# Autodesk Inventor assembly: 240710_case
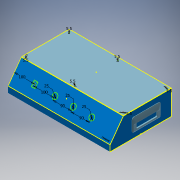
[picture p0: Inventor's stored thumbnail of the model, 180x180]
Saved by Autodesk Inventor 2016 (Build 200138000, 138)
## iProperties
Created: 2024-07-10
Part Number: 240710_case
Material: 일반
Document SubType Name: Assembly
Designer: pc
Author: pc
## Documents named in this file (5)
- D:\CAD_HCH\240710\240710_case.iam
- D:\CAD_HCH\240710\240710_part2.ipt
- D:\CAD_HCH\240710\240710_part3.ipt
- C:\Users\pc\Documents\Inventor\Content Center Files\R2016\ko-KR\ANSI B18.2.3.2M(1)\ANSI B18.2.3.2M - M5x0.8 x 8(2)8.ipt
- D:\CAD_HCH\240711\DR_A-MP200\DR_A-MP200.ipt
## Components (10 placed, 4 different names)
1. 240710_part2:1 — 메이트:1, 플러쉬:1, 플러쉬:2, 메이트:2, 메이트:3
2. 240710_part3:1 — 메이트:1, 플러쉬:1, 플러쉬:2, 삽입:1, 삽입:2, 삽입:3, 삽입:4, 삽입:5, 삽입:6
3. 6각 나사 - 미터 (1) M5x0.8 x 8:1 — 삽입:1
4. 6각 나사 - 미터 (1) M5x0.8 x 8:2 — 삽입:2
5. DR_A-MP200:1 — 메이트:2
6. DR_A-MP200:2 — 메이트:3
7. 6각 나사 - 미터 (1) M5x0.8 x 8:3 — 삽입:3
8. 6각 나사 - 미터 (1) M5x0.8 x 8:4 — 삽입:4
9. 6각 나사 - 미터 (1) M5x0.8 x 8:5 — 삽입:5
10. 6각 나사 - 미터 (1) M5x0.8 x 8:6 — 삽입:6
## Relationships (11: Insert 6, Mate 3, Flush 2)
- 메이트:1 [Mate]: 240710_part2:1 ↔ 240710_part3:1
- 플러쉬:1 [Flush]: 240710_part2:1 ↔ 240710_part3:1
- 플러쉬:2 [Flush]: 240710_part2:1 ↔ 240710_part3:1
- 삽입:1 [Insert]: 240710_part3:1 ↔ 6각 나사 - 미터 (1) M5x0.8 x 8:1
- 삽입:2 [Insert]: 240710_part3:1 ↔ 6각 나사 - 미터 (1) M5x0.8 x 8:2
- 메이트:2 [Mate]: 240710_part2:1 ↔ DR_A-MP200:1
- 삽입:3 [Insert]: 240710_part3:1 ↔ 6각 나사 - 미터 (1) M5x0.8 x 8:3
- 삽입:4 [Insert]: 240710_part3:1 ↔ 6각 나사 - 미터 (1) M5x0.8 x 8:4
- 삽입:5 [Insert]: 240710_part3:1 ↔ 6각 나사 - 미터 (1) M5x0.8 x 8:5
- 삽입:6 [Insert]: 240710_part3:1 ↔ 6각 나사 - 미터 (1) M5x0.8 x 8:6
- 메이트:3 [Mate]: 240710_part2:1 ↔ DR_A-MP200:2
